# Autodesk Inventor assembly: GP8-100
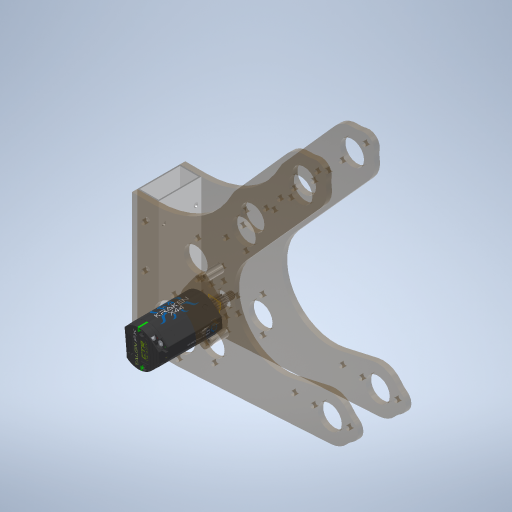
[picture p0: Inventor's stored thumbnail of the model, 512x512]
Saved by Autodesk Inventor 2023.4 (Build 274418000, 418)
## iProperties
Created: 2025-02-26
Part Number: GP8-100
Document SubType Name: Assembly
Designer: dlangdon
Author: dlangdon
## Documents named in this file (8)
- C:\Users\dlangdon\Documents\GitHub\2025-ReefScape---CAD\Gripper\GP8\GP8-100.iam
- C:\Users\dlangdon\Documents\GitHub\2025-ReefScape---CAD\Gripper\GP8\GP8-001.ipt
- C:\Users\dlangdon\Documents\GitHub\2025-ReefScape---CAD\Gripper\GP8\GP8-002.ipt
- C:\Users\dlangdon\Documents\GitHub\2025-ReefScape---CAD\Gripper\GP8\GP8-004.ipt
- C:\Users\dlangdon\Documents\GitHub\2025-ReefScape---CAD\COMMON PARTS\MOTORS\WCP-0941 x44 Kracken.ipt
- C:\Users\dlangdon\Documents\GitHub\2025-ReefScape---CAD\COMMON PARTS\GEARS\32 dp gear\WCP-1464.ipt
- C:\Users\dlangdon\Documents\GitHub\2025-ReefScape---CAD\Gripper\GP6\GP6-006.ipt
- C:\Users\dlangdon\Documents\GitHub\2025-ReefScape---CAD\Gripper\GP8\GP8-003.ipt
## Components (8 placed, 7 different names)
1. GP8-001:1 — Insert:1, Insert:2, Insert:10, Insert:11
2. GP8-002:1 — Insert:3, Insert:4
3. GP8-004:1 — Insert:1, Insert:2, Insert:3, Insert:4
4. GP8-003:1 — Insert:5, Insert:6, Insert:8, Insert:9
5. WCP-0941 x44 Kracken:1 — Insert:5, Insert:6, Insert:7
6. WCP-1464:1 — Insert:7
7. GP6-006:1 — Insert:9, Insert:11
8. GP6-006:2 — Insert:8, Insert:10
## Relationships (11: Insert 11)
- Insert:1: GP8-001:1 ↔ GP8-004:1
- Insert:2: GP8-001:1 ↔ GP8-004:1
- Insert:3: GP8-002:1 ↔ GP8-004:1
- Insert:4: GP8-002:1 ↔ GP8-004:1
- Insert:5: GP8-003:1 ↔ WCP-0941 x44 Kracken:1
- Insert:6: GP8-003:1 ↔ WCP-0941 x44 Kracken:1
- Insert:7: WCP-0941 x44 Kracken:1 ↔ WCP-1464:1
- Insert:8: GP8-003:1 ↔ GP6-006:2
- Insert:9: GP8-003:1 ↔ GP6-006:1
- Insert:10: GP8-001:1 ↔ GP6-006:2
- Insert:11: GP8-001:1 ↔ GP6-006:1
